# Autodesk Inventor assembly: Knobass
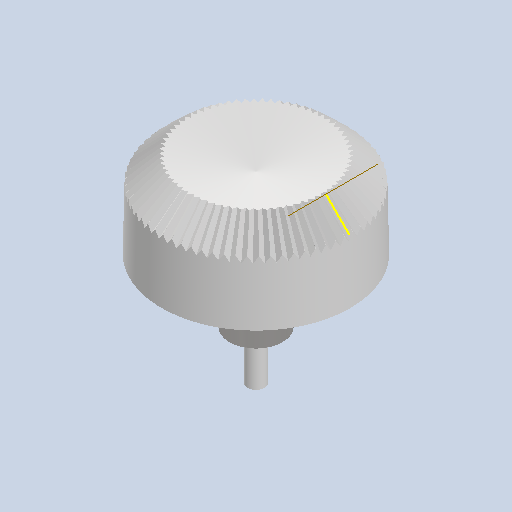
[picture p0: Inventor's stored thumbnail of the model, 512x512]
Saved by Autodesk Inventor 2022 (Build 260153000, 153)
## iProperties
Created: 2023-08-31
Part Number: Knobass
Document SubType Name: Assembly
Designer: THK
Author: THK
## Documents named in this file (5)
- C:\Users\THK\Documents\Inventor\etchasketch\Knobass.iam
- C:\Users\THK\Documents\Inventor\etchasketch\knob.ipt
- C:\Users\THK\Documents\Inventor\etchasketch\Part4.ipt
- C:\Users\THK\Documents\Inventor\Content Center Files\R2022\en-US\BS 290 SKF(30)\BS 290 SKF - SKF 626.ipt
- C:\Users\THK\Documents\Inventor\etchasketch\spacer3.ipt
## Components (5 placed, 4 different names)
1. knob:1 — Flush:1, Flush:2
2. Part4:1 — Flush:1, Mate:1, Mate:2
3. BS 290 SKF 626:1 — Mate:1, Mate:3, Mate:4
4. BS 290 SKF 626:2 — Mate:2, Mate:4
5. spacer3:1 — Flush:2, Mate:3
## Relationships (6: Mate 4, Flush 2)
- Flush:1: knob:1 ↔ Part4:1
- Mate:1: Part4:1 ↔ BS 290 SKF 626:1
- Mate:2: Part4:1 ↔ BS 290 SKF 626:2
- Flush:2: knob:1 ↔ spacer3:1
- Mate:3: BS 290 SKF 626:1 ↔ spacer3:1
- Mate:4 (12 mm): BS 290 SKF 626:1 ↔ BS 290 SKF 626:2
